# Autodesk Inventor assembly: MAINASSEMBLY
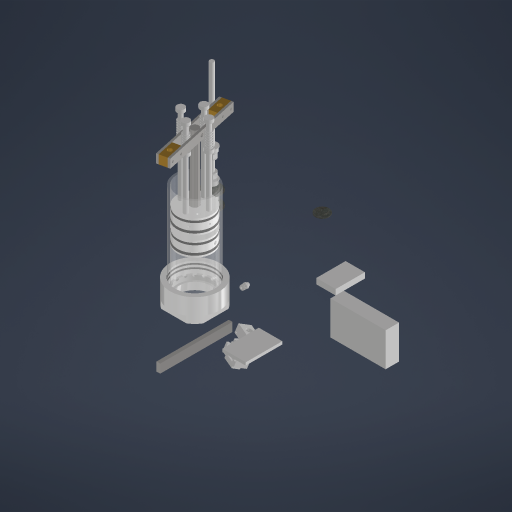
[picture p0: Inventor's stored thumbnail of the model, 512x512]
Saved by Autodesk Inventor 2024 (Build 280153000, 153)
## iProperties
Created: 2025-02-06
Part Number: MAINASSEMBLY
Document SubType Name: Assembly
Designer: Tommy Rohmann
Author: Tommy Rohmann
## Documents named in this file (13)
- C:\Users\Tommy Rohmann\OneDrive\Projects\Microgravity-Press-Washing-Machine\System Design and Documentation\Inventor Design Project\MAINASSEMBLY.iam
- C:\Users\Tommy Rohmann\OneDrive\Projects\Microgravity-Press-Washing-Machine\System Design and Documentation\Inventor Design Project\SUBWashChamber.iam
- C:\Users\Tommy Rohmann\OneDrive\Projects\Microgravity-Press-Washing-Machine\System Design and Documentation\Inventor Design Project\Actuated Ball Valves\SUBBallValve.iam
- C:\Users\Tommy Rohmann\OneDrive\Projects\Microgravity-Press-Washing-Machine\System Design and Documentation\Inventor Design Project\SUBReserviorPiston.iam
- C:\Users\Tommy Rohmann\OneDrive\Projects\Microgravity-Press-Washing-Machine\System Design and Documentation\Inventor Design Project\.25inFittings\5779K109_Push-to-Connect Tube Fitting for Air .ipt
- C:\Users\Tommy Rohmann\OneDrive\Projects\Microgravity-Press-Washing-Machine\System Design and Documentation\Inventor Design Project\SUBFrameBottom.iam
- C:\Users\Tommy Rohmann\OneDrive\Projects\Microgravity-Press-Washing-Machine\System Design and Documentation\Inventor Design Project\SUBDriveShaftACME.iam
- C:\Users\Tommy Rohmann\OneDrive\Projects\Microgravity-Press-Washing-Machine\System Design and Documentation\Inventor Design Project\SUBWashPiston.iam
- C:\Users\Tommy Rohmann\OneDrive\Projects\Microgravity-Press-Washing-Machine\System Design and Documentation\Inventor Design Project\TensionerSprocket.ipt
- C:\Users\Tommy Rohmann\OneDrive\Projects\Microgravity-Press-Washing-Machine\System Design and Documentation\Inventor Design Project\SUBWashThrustArm.iam
- C:\Users\Tommy Rohmann\OneDrive\Projects\Microgravity-Press-Washing-Machine\System Design and Documentation\Inventor Design Project\ElectricalFixtures\LCDScreen.ipt
- C:\Users\Tommy Rohmann\OneDrive\Projects\Microgravity-Press-Washing-Machine\System Design and Documentation\Inventor Design Project\ElectricalFixtures\PowerSupply.ipt
- C:\Users\Tommy Rohmann\OneDrive\Projects\Microgravity-Press-Washing-Machine\System Design and Documentation\Inventor Design Project\ElectricalFixtures\RaspberryPi.ipt
## Components (12 placed, 12 different names)
1. SUBWashChamber:1 [sub-assembly] — Mate:1, Tangent:1, Mate:4, Mate:5, Mate:9, Mate:12
2. SUBBallValve:1 [sub-assembly]
3. SUBReserviorPiston:1 [sub-assembly] — Mate:4
4. 5779K109_Push-to-Connect Tube Fitting for Air :1 — Mate:1, Tangent:1
5. SUBFrameBottom:1 [sub-assembly] — Mate:9, Mate:12
6. SUBWashPiston:1 [sub-assembly] — Mate:5, Mate:6, Flush:1, Tangent:2
7. TensionerSprocket:1
8. SUBWashThrustArm:1 [sub-assembly] — Mate:6, Flush:1, Tangent:2, Mate:21
9. LCDScreen:1
10. PowerSupply:1
11. RaspberryPi:1
12. SUBDriveShaftACME:4 [sub-assembly] — Mate:21
## Relationships (10: Mate 7, Tangent 2, Flush 1)
- Mate:1: SUBWashChamber:1 ↔ 5779K109_Push-to-Connect Tube Fitting for Air :1
- Tangent:1 (10.16 mm): SUBWashChamber:1 ↔ 5779K109_Push-to-Connect Tube Fitting for Air :1
- Mate:4: SUBWashChamber:1 ↔ SUBReserviorPiston:1
- Mate:5: SUBWashChamber:1 ↔ SUBWashPiston:1
- Mate:6: SUBWashPiston:1 ↔ SUBWashThrustArm:1
- Flush:1: SUBWashPiston:1 ↔ SUBWashThrustArm:1
- Tangent:2: SUBWashPiston:1 ↔ SUBWashThrustArm:1
- Mate:9: SUBWashChamber:1 ↔ SUBFrameBottom:1
- Mate:12: SUBWashChamber:1 ↔ SUBFrameBottom:1
- Mate:21: SUBWashThrustArm:1 ↔ SUBDriveShaftACME:4
